# Autodesk Inventor assembly: ASY MSC 202 LEFT BOARD
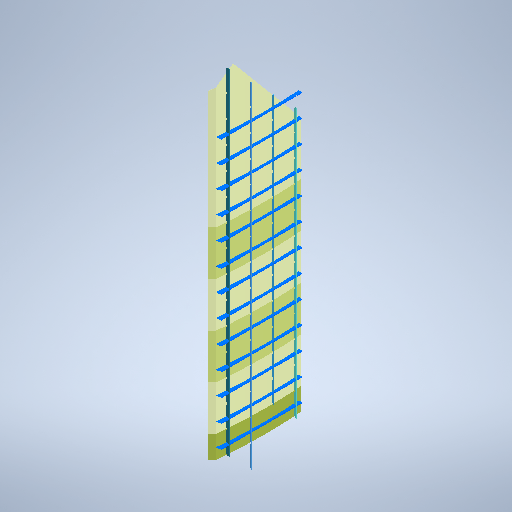
[picture p0: Inventor's stored thumbnail of the model, 512x512]
Saved by Autodesk Inventor 2025 (Build 290162010, 162A)
## iProperties
Created: 2024-07-21
Part Number: ASY MSC 202 LEFT BOARD
Document SubType Name: Assembly
Designer: pokla
Author: pokla
## Documents named in this file (10)
- C:\Users\user\YandexDisk\домашниий пк\Inventor\Manturovo\Manturovo_Se-clar\ASY MSC 202 LEFT BOARD.iam
- C:\Users\user\YandexDisk\домашниий пк\Inventor\Manturovo\Manturovo_Se-clar\MSC 052 rib board.ipt
- C:\Users\user\YandexDisk\домашниий пк\Inventor\Manturovo\Manturovo_Se-clar\MSC 024 sheet board main.ipt
- C:\Users\user\YandexDisk\домашниий пк\Inventor\Manturovo\Manturovo_Se-clar\MSC 023 sheet board.ipt
- C:\Users\user\YandexDisk\домашниий пк\Inventor\Manturovo\Manturovo_Se-clar\MSC 063 stringer board #.ipt
- C:\Users\user\YandexDisk\домашниий пк\Inventor\Manturovo\Manturovo_Se-clar\MSC 064 stringer board ##.ipt
- C:\Users\user\YandexDisk\домашниий пк\Inventor\Manturovo\Manturovo_Se-clar\MSC 065 stringer board ###.ipt
- C:\Users\user\YandexDisk\домашниий пк\Inventor\Manturovo\Manturovo_Se-clar\MSC 066 stringer board ####.ipt
- C:\Users\user\YandexDisk\домашниий пк\Inventor\Manturovo\Manturovo_Se-clar\MSC 025 sheet board withers 1.ipt
- C:\Users\user\YandexDisk\домашниий пк\Inventor\Manturovo\Manturovo_Se-clar\MSC 027 sheet board face 1.ipt
## Components (39 placed, 14 different names)
1. MSC 052 rib board.ipt:3 — Rigid:16, Flush:1, Flush:2, Flush:3
2. MSC 024 sheet board main.ipt:1 — Rigid:19
3. MSC 024 sheet board main.ipt:2
4. MSC 024 sheet board main.ipt:3
5. MSC 024 sheet board main.ipt:4
6. MSC 024 sheet board main.ipt:5
7. MSC 023 sheet board.ipt:1 — Flush:1, Flush:2, Flush:3, Rigid:19
8. MSC 065 stringer board ###.ipt:2
9. MSC 066 stringer board ####.ipt:2
10. MSC 025 sheet board withers 1.ipt:1
11. MSC 027 sheet board face 1.ipt:1
12. MSC 052 rib board.ipt:5 — Rigid:16, Rigid:20
13. MSC 063 stringer board #.ipt:3 — Rigid:41
14. MSC 064 stringer board ##.ipt:3 — Rigid:38
15. MSC 065 stringer board ###.ipt:3 — Rigid:35
16. MSC 066 stringer board ####.ipt:3 — Rigid:32
17. MSC 052 rib board:4 — Rigid:20, Rigid:21
18. MSC 052 rib board:6 — Rigid:21, Rigid:22
19. MSC 052 rib board:7 — Rigid:22, Rigid:25
20. MSC 052 rib board:8 — Rigid:25
21. MSC 052 rib board:9
22. MSC 052 rib board:10 — Rigid:31
23. MSC 052 rib board:11 — Rigid:31
24. MSC 052 rib board:12
25. MSC 052 rib board:13
26. MSC 052 rib board:14
27. MSC 052 rib board:15
28. МОО 056 стрингер борт 6:4 — Rigid:32, Rigid:33
29. МОО 056 стрингер борт 6:5 — Rigid:33, Rigid:34
30. МОО 056 стрингер борт 6:6 — Rigid:34
31. МОО 055 стрингер борт 5:4 — Rigid:35, Rigid:36
32. МОО 055 стрингер борт 5:5 — Rigid:36, Rigid:37
33. МОО 055 стрингер борт 5:6 — Rigid:37
34. МОО 054 стрингер борт 4:4 — Rigid:38, Rigid:39
35. МОО 054 стрингер борт 4:5 — Rigid:39, Rigid:40
36. МОО 054 стрингер борт 4:6 — Rigid:40
37. МОО 053 стрингер борт 3:4 — Rigid:41, Rigid:42
38. МОО 053 стрингер борт 3:5 — Rigid:42, Rigid:43
39. МОО 053 стрингер борт 3:6 — Rigid:43
## Relationships (40: WeldJoint 36, Flush 3, Mate 1)
- [WeldJoint]: MSC 024 sheet board main.ipt:1 ↔ MSC 024 sheet board main.ipt:2
- [WeldJoint]: MSC 024 sheet board main.ipt:2 ↔ MSC 024 sheet board main.ipt:3
- [WeldJoint]: MSC 024 sheet board main.ipt:3 ↔ MSC 024 sheet board main.ipt:4
- [WeldJoint]: MSC 024 sheet board main.ipt:4 ↔ MSC 024 sheet board main.ipt:5
- [Mate]: MSC 024 sheet board main.ipt:1 ↔ MSC 023 sheet board.ipt:1
- [WeldJoint]: MSC 024 sheet board main.ipt:5 ↔ MSC 025 sheet board withers 1.ipt:1
- [WeldJoint]: MSC 025 sheet board withers 1.ipt:1 ↔ MSC 027 sheet board face 1.ipt:1
- [WeldJoint] (2 mm): MSC 052 rib board.ipt:3 ↔ MSC 066 stringer board ####.ipt:2
- [WeldJoint]: MSC 065 stringer board ###.ipt:2 ↔ MSC 065 stringer board ###.ipt:3
- [WeldJoint]: MSC 066 stringer board ####.ipt:2 ↔ MSC 066 stringer board ####.ipt:3
- [WeldJoint] (2 mm): MSC 052 rib board.ipt:3 ↔ MSC 065 stringer board ###.ipt:2
- [WeldJoint] (2 mm): MSC 052 rib board.ipt:3 ↔ MSC 063 stringer board #.ipt:3
- Rigid:16 [WeldJoint] (-500 mm): MSC 052 rib board.ipt:3 ↔ MSC 052 rib board.ipt:5
- Flush:1 (248 mm): MSC 052 rib board.ipt:3 ↔ MSC 023 sheet board.ipt:1
- Flush:2: MSC 052 rib board.ipt:3 ↔ MSC 023 sheet board.ipt:1
- Flush:3: MSC 052 rib board.ipt:3 ↔ MSC 023 sheet board.ipt:1
- Rigid:19 [WeldJoint]: MSC 024 sheet board main.ipt:1 ↔ MSC 023 sheet board.ipt:1
- Rigid:20 [WeldJoint] (-500 mm): MSC 052 rib board.ipt:5 ↔ MSC 052 rib board:4
- Rigid:21 [WeldJoint] (-500 mm): MSC 052 rib board:4 ↔ MSC 052 rib board:6
- Rigid:22 [WeldJoint] (-500 mm): MSC 052 rib board:6 ↔ MSC 052 rib board:7
- [WeldJoint] (-500 mm): MSC 052 rib board:8 ↔ MSC 052 rib board:9
- [WeldJoint] (-500 mm): MSC 052 rib board:9 ↔ MSC 052 rib board:10
- Rigid:25 [WeldJoint] (-500 mm): MSC 052 rib board:7 ↔ MSC 052 rib board:8
- [WeldJoint] (-500 mm): MSC 052 rib board:11 ↔ MSC 052 rib board:12
- [WeldJoint] (-500 mm): MSC 052 rib board:12 ↔ MSC 052 rib board:13
- [WeldJoint] (-500 mm): MSC 052 rib board:14 ↔ MSC 052 rib board:15
- [WeldJoint] (-500 mm): MSC 052 rib board:13 ↔ MSC 052 rib board:14
- Rigid:31 [WeldJoint] (-500 mm): MSC 052 rib board:10 ↔ MSC 052 rib board:11
- Rigid:32 [WeldJoint]: MSC 066 stringer board ####.ipt:3 ↔ МОО 056 стрингер борт 6:4
- Rigid:33 [WeldJoint]: МОО 056 стрингер борт 6:4 ↔ МОО 056 стрингер борт 6:5
- Rigid:34 [WeldJoint]: МОО 056 стрингер борт 6:5 ↔ МОО 056 стрингер борт 6:6
- Rigid:35 [WeldJoint]: MSC 065 stringer board ###.ipt:3 ↔ МОО 055 стрингер борт 5:4
- Rigid:36 [WeldJoint]: МОО 055 стрингер борт 5:4 ↔ МОО 055 стрингер борт 5:5
- Rigid:37 [WeldJoint]: МОО 055 стрингер борт 5:5 ↔ МОО 055 стрингер борт 5:6
- Rigid:38 [WeldJoint]: MSC 064 stringer board ##.ipt:3 ↔ МОО 054 стрингер борт 4:4
- Rigid:39 [WeldJoint]: МОО 054 стрингер борт 4:4 ↔ МОО 054 стрингер борт 4:5
- Rigid:40 [WeldJoint]: МОО 054 стрингер борт 4:5 ↔ МОО 054 стрингер борт 4:6
- Rigid:41 [WeldJoint]: MSC 063 stringer board #.ipt:3 ↔ МОО 053 стрингер борт 3:4
- Rigid:42 [WeldJoint]: МОО 053 стрингер борт 3:4 ↔ МОО 053 стрингер борт 3:5
- Rigid:43 [WeldJoint]: МОО 053 стрингер борт 3:5 ↔ МОО 053 стрингер борт 3:6
